# Autodesk Inventor assembly: Fox_Plus_Robinson
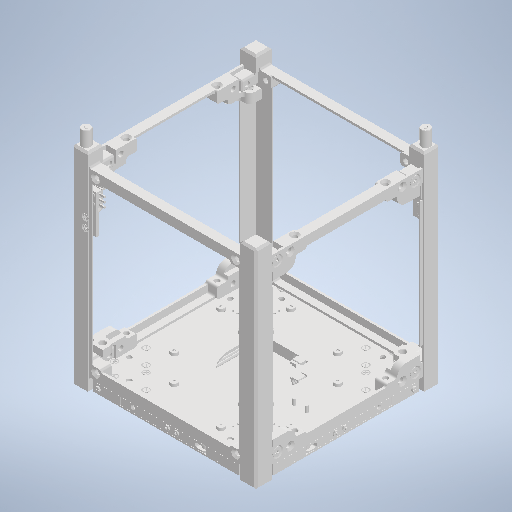
[picture p0: Inventor's stored thumbnail of the model, 512x512]
Saved by Autodesk Inventor 2025 (Build 290162000, 162)
## iProperties
Created: 2024-03-31
Part Number: Fox_Plus_Robinson
Document SubType Name: Assembly
Designer: arobi
Author: arobi
## Documents named in this file (3)
- C:\Users\arobi\Documents\AMSAT\Fox-Plus\Model\Fox_Plus_Robinson.iam
- C:\Users\arobi\Documents\AMSAT\Fox-Plus\Model\ISIS CubeSat STS PC104 Skeleton.iam
- C:\Users\arobi\Documents\AMSAT\Fox-Plus\Model\ISIS_ANTS1_REVD_STEP_STOWED_asm.iam
## Components (2 placed, 2 different names)
1. ISIS CubeSat STS PC104 Skeleton:1 [sub-assembly] — Mate:4, Flush:2, Flush:1, Mate:1, Mate:2, Mate:3
2. ISIS_ANTS1_REVD_STEP_STOWED_asm:1 [sub-assembly] — Mate:1, Mate:2, Mate:3
## Relationships (6: Mate 4, Flush 2)
- Mate:4: ISIS CubeSat STS PC104 Skeleton:1
- Flush:2: ISIS CubeSat STS PC104 Skeleton:1
- Flush:1: ISIS CubeSat STS PC104 Skeleton:1
- Mate:1: ISIS CubeSat STS PC104 Skeleton:1 ↔ ISIS_ANTS1_REVD_STEP_STOWED_asm:1
- Mate:2: ISIS CubeSat STS PC104 Skeleton:1 ↔ ISIS_ANTS1_REVD_STEP_STOWED_asm:1
- Mate:3: ISIS CubeSat STS PC104 Skeleton:1 ↔ ISIS_ANTS1_REVD_STEP_STOWED_asm:1
